# Autodesk Inventor assembly: roll_support_behind_v1
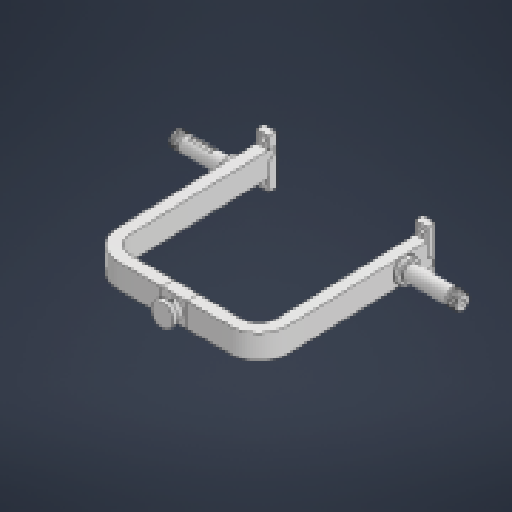
[picture p0: Inventor's stored thumbnail of the model, 512x512]
Saved by Autodesk Inventor 2026.1 (Build 301233020, 233B)
## iProperties
Created: 2025-12-01
Part Number: roll_support_behind_v1
Document SubType Name: Assembly
Designer: jaewook
Author: jaewook
## Documents named in this file (4)
- C:\Users\kjh19\Documents\Inventor\project\final\roll_support_behind_v1.iam
- C:\Users\kjh19\Documents\Inventor\project\proto2\example\솔리드6.ipt
- C:\Users\kjh19\Documents\Inventor\project\final\stopper.ipt
- C:\Users\kjh19\Documents\Inventor\project\final\rotion_stopper.ipt
## Components (3 placed, 3 different names)
1. 솔리드6:1 — 메이트:1, 메이트:2
2. stopper:1 — 메이트:1, 메이트:2
3. rotion_stopper:1
## Relationships (2: Mate 2)
- 메이트:1 [Mate]: 솔리드6:1 ↔ stopper:1
- 메이트:2 [Mate]: 솔리드6:1 ↔ stopper:1
